# Autodesk Inventor assembly: HubPVCHoleJig
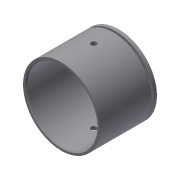
[picture p0: Inventor's stored thumbnail of the model, 180x180]
Saved by Autodesk Inventor 2017 (Build 210142000, 142)
## iProperties
Created: 2017-02-15
Part Number: HubPVCHoleJig
Document SubType Name: Assembly
Designer: krosie
Author: krosie
## Documents named in this file (3)
- C:\Users\krosie\Google Drive\HERA\hera-cad\jigs\HubPVCHoleJig.iam
- C:\Users\krosie\Google Drive\HERA\hera-cad\jigs\HubSparHole.ipt
- C:\Users\krosie\Google Drive\HERA\hera-cad\jigs\HubSparPlate.ipt
## Components (2 placed, 2 different names)
1. HubSparHole:1 — Flush:1
2. HubSparPlate:1 — Flush:1
## Relationships (1: Flush 1)
- Flush:1: HubSparHole:1 ↔ HubSparPlate:1
